# Autodesk Inventor assembly: Korp
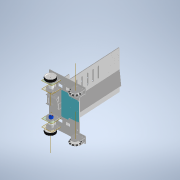
[picture p0: Inventor's stored thumbnail of the model, 180x180]
Saved by Autodesk Inventor 2021.1 (Build 251245010, 245A)
## iProperties
Created: 2023-03-13
Part Number: Korp
Document SubType Name: Assembly
Designer: User
Author: User
## Documents named in this file (13)
- C:\Users\User\Documents\Savka\3d\Korp.iam
- C:\Users\User\Documents\Savka\3d\Korpus.ipt
- C:\Users\User\Documents\Savka\3d\Korpus 2.ipt
- C:\Users\User\Documents\Savka\3d\Korpus 3.ipt
- C:\Users\User\Documents\Savka\3d\Импорт\36466_txm-4 inch omni wheel.ipt
- C:\Users\User\Documents\Savka\3d\Korpus 4.ipt
- C:\Users\User\Documents\Savka\3d\Korpus 5.ipt
- C:\Users\User\Documents\Savka\3d\Импорт\44260_txm torquenado dc motor.ipt
- C:\Users\User\Documents\Savka\3d\Деталь1.ipt
- C:\Users\User\Documents\Savka\3d\Korpus 6.ipt
- C:\Users\User\Documents\Savka\3d\Импорт\39055_txm-4 inch wheel.ipt
- C:\Users\User\Documents\Savka\3d\Импорт\корпус.ipt
- C:\Users\User\Documents\Savka\3d\Импорт\Platforma_kolesa.ipt
## Components (21 placed, 12 different names)
1. Korpus:1 — Заподлицо:1, Заподлицо:4, Заподлицо:9
2. Korpus 2:1 — Заподлицо:1, Заподлицо:2
3. Korpus 3:1 — Заподлицо:2, Заподлицо:3, Заподлицо:5, Совмещение:2, Совмещение:3, Заподлицо:6, Заподлицо:7, Совмещение:4, Совмещение:5, Совмещение:6, Совмещение:7, Заподлицо:8, Заподлицо:10, Угол:1, Заподлицо:14, Совмещение:12, Совмещение:13, Заподлицо:15, Совмещение:14, Совмещение:15, Угол:2, Угол:4, Совмещение:19, Заподлицо:17, Угол:5, Совмещение:21, Заподлицо:18, Совмещение:27, Совмещение:28, Заподлицо:19, Совмещение:29, Совмещение:33, Заподлицо:20
4. 36466_txm-4 inch omni wheel:2 — Совмещение:10, Совмещение:32
5. Korpus 4:1 — Заподлицо:3, Заподлицо:4, Совмещение:31, Совмещение:33
6. Korpus 4:2 — Заподлицо:5, Совмещение:2, Совмещение:3, Совмещение:22, Совмещение:24, Совмещение:25, Совмещение:30, Заподлицо:20
7. Korpus 4:3 — Заподлицо:7, Совмещение:4, Совмещение:6, Совмещение:10
8. Korpus 4:4 — Заподлицо:6, Совмещение:5, Совмещение:7, Совмещение:27, Совмещение:32
9. Korpus 5:1 — Заподлицо:8, Заподлицо:9, Совмещение:8, Совмещение:9, Заподлицо:12
10. 44260_txm torquenado dc motor:1 — Совмещение:8, Совмещение:9, Угол:1, Заподлицо:13, Совмещение:11
11. Деталь1:1 — Заподлицо:10, Заподлицо:11, Совмещение:20
12. Korpus 6:1 — Заподлицо:11, Заподлицо:12
13. 39055_txm-4 inch wheel:1 — Заподлицо:13, Совмещение:11
14. Korpus 5:2 — Заподлицо:14, Совмещение:12, Совмещение:13, Угол:3, Совмещение:16, Совмещение:17, Совмещение:18
15. Деталь1:2 — Заподлицо:15, Совмещение:14, Совмещение:15
16. 44260_txm torquenado dc motor:2 — Угол:2, Угол:3, Совмещение:16, Совмещение:17, Заподлицо:16
17. 39055_txm-4 inch wheel:2 — Совмещение:18, Заподлицо:16
18. корпус:1 — Угол:4, Совмещение:19, Заподлицо:17, Совмещение:20
19. Platforma_kolesa:1 — Угол:5, Совмещение:21, Заподлицо:18, Совмещение:22, Совмещение:24, Совмещение:25
20. Korpus 6:2 — Совмещение:28, Заподлицо:19, Совмещение:29
21. 36466_txm-4 inch omni wheel:3 — Совмещение:30, Совмещение:31
## Relationships (55: Mate 30, Flush 20, Angle 5)
- Заподлицо:1 [Flush]: Korpus:1 ↔ Korpus 2:1
- Заподлицо:2 [Flush]: Korpus 2:1 ↔ Korpus 3:1
- Заподлицо:3 [Flush]: Korpus 3:1 ↔ Korpus 4:1
- Заподлицо:4 [Flush]: Korpus:1 ↔ Korpus 4:1
- Заподлицо:5 [Flush]: Korpus 3:1 ↔ Korpus 4:2
- Совмещение:2 [Mate]: Korpus 3:1 ↔ Korpus 4:2
- Совмещение:3 [Mate]: Korpus 3:1 ↔ Korpus 4:2
- Заподлицо:6 [Flush]: Korpus 3:1 ↔ Korpus 4:4
- Заподлицо:7 [Flush]: Korpus 3:1 ↔ Korpus 4:3
- Совмещение:4 [Mate]: Korpus 3:1 ↔ Korpus 4:3
- Совмещение:5 [Mate]: Korpus 3:1 ↔ Korpus 4:4
- Совмещение:6 [Mate]: Korpus 3:1 ↔ Korpus 4:3
- Совмещение:7 [Mate]: Korpus 3:1 ↔ Korpus 4:4
- Заподлицо:8 [Flush]: Korpus 3:1 ↔ Korpus 5:1
- Заподлицо:9 [Flush]: Korpus:1 ↔ Korpus 5:1
- Совмещение:8 [Mate]: Korpus 5:1 ↔ 44260_txm torquenado dc motor:1
- Совмещение:9 [Mate]: Korpus 5:1 ↔ 44260_txm torquenado dc motor:1
- Заподлицо:10 [Flush]: Korpus 3:1 ↔ Деталь1:1
- Угол:1 [Angle] (0 deg): Korpus 3:1 ↔ 44260_txm torquenado dc motor:1
- Совмещение:10 [Mate]: 36466_txm-4 inch omni wheel:2 ↔ Korpus 4:3
- Заподлицо:11 [Flush]: Деталь1:1 ↔ Korpus 6:1
- Заподлицо:12 [Flush]: Korpus 5:1 ↔ Korpus 6:1
- Заподлицо:13 [Flush]: 44260_txm torquenado dc motor:1 ↔ 39055_txm-4 inch wheel:1
- Совмещение:11 [Mate]: 44260_txm torquenado dc motor:1 ↔ 39055_txm-4 inch wheel:1
- Заподлицо:14 [Flush]: Korpus 3:1 ↔ Korpus 5:2
- Совмещение:12 [Mate]: Korpus 3:1 ↔ Korpus 5:2
- Совмещение:13 [Mate]: Korpus 3:1 ↔ Korpus 5:2
- Заподлицо:15 [Flush]: Korpus 3:1 ↔ Деталь1:2
- Совмещение:14 [Mate]: Korpus 3:1 ↔ Деталь1:2
- Совмещение:15 [Mate]: Korpus 3:1 ↔ Деталь1:2
- Угол:2 [Angle] (0 deg): Korpus 3:1 ↔ 44260_txm torquenado dc motor:2
- Угол:3 [Angle] (0 deg): Korpus 5:2 ↔ 44260_txm torquenado dc motor:2
- Совмещение:16 [Mate]: Korpus 5:2 ↔ 44260_txm torquenado dc motor:2
- Совмещение:17 [Mate]: Korpus 5:2 ↔ 44260_txm torquenado dc motor:2
- Совмещение:18 [Mate]: Korpus 5:2 ↔ 39055_txm-4 inch wheel:2
- Заподлицо:16 [Flush]: 44260_txm torquenado dc motor:2 ↔ 39055_txm-4 inch wheel:2
- Угол:4 [Angle] (0 deg): Korpus 3:1 ↔ корпус:1
- Совмещение:19 [Mate]: Korpus 3:1 ↔ корпус:1
- Заподлицо:17 [Flush]: Korpus 3:1 ↔ корпус:1
- Совмещение:20 [Mate] (70.943 mm): Деталь1:1 ↔ корпус:1
- Угол:5 [Angle] (0 deg): Korpus 3:1 ↔ Platforma_kolesa:1
- Совмещение:21 [Mate]: Korpus 3:1 ↔ Platforma_kolesa:1
- Заподлицо:18 [Flush]: Korpus 3:1 ↔ Platforma_kolesa:1
- Совмещение:22 [Mate] (119.463 mm): Korpus 4:2 ↔ Platforma_kolesa:1
- Совмещение:24 [Mate] (110 mm): Korpus 4:2 ↔ Platforma_kolesa:1
- Совмещение:25 [Mate] (110 mm): Korpus 4:2 ↔ Platforma_kolesa:1
- Совмещение:27 [Mate]: Korpus 3:1 ↔ Korpus 4:4
- Совмещение:28 [Mate]: Korpus 3:1 ↔ Korpus 6:2
- Заподлицо:19 [Flush]: Korpus 3:1 ↔ Korpus 6:2
- Совмещение:29 [Mate]: Korpus 3:1 ↔ Korpus 6:2
- Совмещение:30 [Mate]: Korpus 4:2 ↔ 36466_txm-4 inch omni wheel:3
- Совмещение:31 [Mate] (4 mm): Korpus 4:1 ↔ 36466_txm-4 inch omni wheel:3
- Совмещение:32 [Mate] (4 mm): 36466_txm-4 inch omni wheel:2 ↔ Korpus 4:4
- Совмещение:33 [Mate]: Korpus 3:1 ↔ Korpus 4:1
- Заподлицо:20 [Flush]: Korpus 3:1 ↔ Korpus 4:2
